# Autodesk Inventor assembly: Assembly1
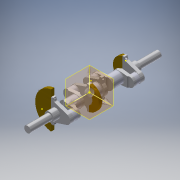
[picture p0: Inventor's stored thumbnail of the model, 180x180]
Saved by Autodesk Inventor 2019 (Build 230136000, 136)
## iProperties
Created: 2019-06-29
Part Number: Assembly1
Document SubType Name: Assembly
Designer: usuario
Mass: 181.192 g
Surface Area: 482.745 cm^2
Volume: 172.255 cm^3
Density: 1.05188 g/cm^3
Author: usuario
## Documents named in this file (6)
- E:\OSCAR\UNAL\6to SEMESTRE\Principios de dinámica\Proyectos\Proyecto 2\Mio\Assembly1.iam
- E:\OSCAR\UNAL\6to SEMESTRE\Principios de dinámica\Proyectos\Proyecto 2\Mio\cigueñal.ipt
- E:\OSCAR\UNAL\6to SEMESTRE\Principios de dinámica\Proyectos\Proyecto 2\Mio\Contrapeso2.ipt
- E:\OSCAR\UNAL\6to SEMESTRE\Principios de dinámica\Proyectos\Proyecto 2\Mio\ContrapesoGrande1.ipt
- E:\OSCAR\UNAL\6to SEMESTRE\Principios de dinámica\Proyectos\Proyecto 2\Mio\Pasador.ipt
- E:\OSCAR\UNAL\6to SEMESTRE\Principios de dinámica\Proyectos\Proyecto 2\Mio\Contrapeso1.ipt
## Components (6 placed, 5 different names)
1. cigueñal:1 — Rigid:1, Rigid:2, Insert:1, Rotational:1
2. ContrapesoGrande1:1 — Rigid:1, Insert:2
3. Contrapeso2:1 — Rigid:2
4. Pasador:1 — Insert:1
5. Pasador:2 — Insert:2
6. Contrapeso1:1 — Rotational:1
## Relationships (5: WeldJoint 2, Insert 2, RevoluteJoint 1)
- Rigid:1 [WeldJoint]: cigueñal:1 ↔ ContrapesoGrande1:1
- Rigid:2 [WeldJoint]: cigueñal:1 ↔ Contrapeso2:1
- Insert:1 (-6 mm): cigueñal:1 ↔ Pasador:1
- Insert:2 (-30 mm): ContrapesoGrande1:1 ↔ Pasador:2
- Rotational:1 [RevoluteJoint]: cigueñal:1 ↔ Contrapeso1:1
